# Autodesk Inventor assembly: Assembly6
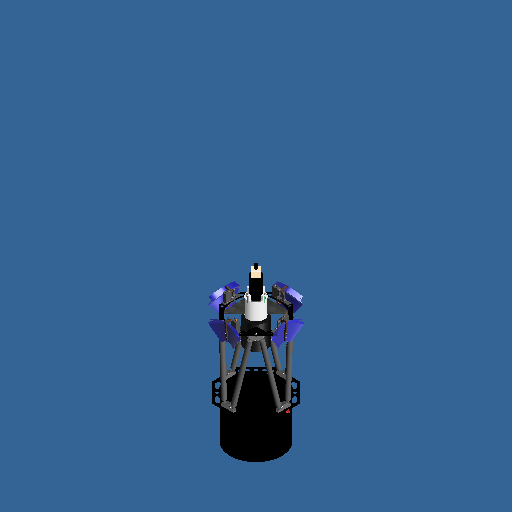
[picture p0: Inventor's stored thumbnail of the model, 512x512]
Saved by Autodesk Inventor 2026.2 (Build 302298000, 298)
## iProperties
Created: 2025-12-09
Part Number: Assembly6
Document SubType Name: Assembly
Designer: Thoma
Mass: 27295.5 g
Surface Area: 25498 cm^2
Volume: 10830.6 cm^3
Density: 2.52023 g/cm^3
Author: Thoma
## Documents named in this file (39)
- C:\Users\Thoma\OneDrive\Desktop\dir\telescope_cover\main\version_2\Main_v5.iam
- C:\Users\Thoma\OneDrive\Desktop\dir\telescope_cover\telescope\version_3\Telescope_End.ipt
- C:\Users\Thoma\OneDrive\Desktop\dir\telescope_cover\telescope\version_3\Triangle.ipt
- C:\Users\Thoma\OneDrive\Desktop\dir\telescope_cover\telescope\version_3\Triangle_Bracket_Top.ipt
- C:\Users\Thoma\OneDrive\Desktop\dir\telescope_cover\telescope\version_3\Carbon_Fibre.ipt
- C:\Users\Thoma\OneDrive\Desktop\dir\telescope_cover\telescope\version_3\5mm Screw.ipt
- C:\Users\Thoma\OneDrive\Desktop\dir\telescope_cover\telescope\version_3\35mm_bolt.ipt
- C:\Users\Thoma\OneDrive\Desktop\dir\telescope_cover\telescope\version_3\Triangle_Bracket_Bottom_MIR.ipt
- C:\Users\Thoma\OneDrive\Desktop\dir\telescope_cover\telescope\version_3\Telescope_Base.ipt
- C:\Users\Thoma\OneDrive\Desktop\dir\telescope_cover\telescope\version_3\Full_shaft_Simplify_3.ipt
- C:\Users\Thoma\OneDrive\Desktop\dir\telescope_cover\telescope\version_3\30mm_bolt.ipt
- C:\Users\Thoma\OneDrive\Desktop\dir\telescope_cover\telescope\version_3\Baffle.ipt
- C:\Users\Thoma\OneDrive\Desktop\dir\telescope_cover\telescope\version_3\Bottom_End_Top.ipt
- C:\Users\Thoma\OneDrive\Desktop\dir\telescope_cover\telescope\version_3\Laser.ipt
- C:\Users\Thoma\OneDrive\Desktop\dir\telescope_cover\cover\central_cover_v1.ipt
- C:\Users\Thoma\OneDrive\Desktop\dir\telescope_cover\cover\base_plate_v11.ipt
- C:\Users\Thoma\OneDrive\Desktop\dir\telescope_cover\cover\base_plate_bottom_v5.ipt
- C:\Users\Thoma\OneDrive\Documents\Inventor\Content Center Files\R2026\en-US\ISO 4035(2)\ISO 4035 - M4 - ISO.ipt
- C:\Users\Thoma\OneDrive\Desktop\dir\telescope_cover\servo\DSS-M15S Servo.ipt
- C:\Users\Thoma\OneDrive\Documents\Inventor\Content Center Files\R2026\en-US\ISO 4762(2)\ISO 4762 - M4 x 16ISO.ipt
- C:\Users\Thoma\OneDrive\Desktop\dir\telescope_cover\cover\pawn_v3.ipt
- C:\Users\Thoma\OneDrive\Documents\Inventor\Content Center Files\R2026\en-US\DIN 6796\DIN 6796 - 2.ipt
- C:\Users\Thoma\OneDrive\Documents\Inventor\Content Center Files\R2026\en-US\DIN 912\DIN 912 - M2 x 0.4 x 8 x 7.ipt
- C:\Users\Thoma\OneDrive\Documents\Inventor\Content Center Files\R2026\en-US\DIN 912\DIN 912 - M2 x 0.4 x 5 x 4.ipt
- C:\Users\Thoma\OneDrive\Desktop\dir\telescope_cover\cover\rod_v11.ipt
- C:\Users\Thoma\OneDrive\Documents\Inventor\Content Center Files\R2026\en-US\ISO 7092\ISO 7092 - ST 4 - 140 HV.ipt
- C:\Users\Thoma\OneDrive\Desktop\dir\telescope_cover\cover\Cover_Upper_v5.ipt
- C:\Users\Thoma\OneDrive\Desktop\dir\telescope_cover\cover\4mm_washer_1mm.ipt
- C:\Users\Thoma\OneDrive\Documents\Inventor\Content Center Files\R2026\en-US\ISO 4762(2)\ISO 4762 - M4 x 20ISO.ipt
- C:\Users\Thoma\OneDrive\Documents\Inventor\Content Center Files\R2026\en-US\ISO 4032(2)\ISO 4032 - M4 - ISO.ipt
- C:\Users\Thoma\OneDrive\Documents\Inventor\Content Center Files\R2026\en-US\ISO 7093 A\ISO 7093 A - ST 4 - 140 HV .ipt
- C:\Users\Thoma\OneDrive\Documents\Inventor\Content Center Files\R2026\en-US\ISO 4762(2)\ISO 4762 - M4 x 30ISO.ipt
- C:\Users\Thoma\OneDrive\Desktop\dir\telescope_cover\servo\limit_switch_v2.ipt
- C:\Users\Thoma\OneDrive\Documents\Inventor\Content Center Files\R2026\en-US\ISO 7089\ISO 7089 - 4 - 140 HV(1).ipt
- C:\Users\Thoma\OneDrive\Desktop\dir\telescope_cover\cover\base_plate_v12.ipt
- C:\Users\Thoma\OneDrive\Documents\Inventor\Content Center Files\R2026\en-US\ISO 7089\ISO 7089 - 2 - 140 HV(1).ipt
- C:\Users\Thoma\OneDrive\Documents\Inventor\Content Center Files\R2026\en-US\ISO 4762(2)\ISO 4762 - M2 x 8ISO.ipt
- C:\Users\Thoma\OneDrive\Desktop\dir\telescope_cover\cover\Cover_Lower_v5.ipt
- C:\Users\Thoma\OneDrive\Desktop\dir\telescope_cover\screws\M4 Washer - 9.0 x 0.9 - Black\M4 Washer - 9.0 x 0.9 - Black\M4 Washer - 9.0 x 0.9 - Black.ipt
## Components (238 placed, 38 different names)
1. Laser:2 — Mate:214, Flush:220, Flush:221
2. Laser:1 — Mate:215, Flush:218, Flush:219
3. Baffle:1 — Mate:83
4. Carbon_Fibre:1 — Mate:7, Mate:11, Flush:1, Mate:12, Mate:13, Mate:14, Mate:15, Mate:62, Mate:83, Mate:92, Mate:93, Mate:96, Mate:97, Mate:98, Mate:100, Mate:123, Mate:124, Mate:125, Mate:213, Mate:220, Angle:84, Flush:223, Flush:224, Flush:225, Flush:226
5. Telescope_Base:1 — Mate:62, Angle:31, Mate:89, Mate:90, Angle:40, Mate:108, Mate:109, Angle:48, Mate:110, Mate:111, Angle:49, Mate:112, Mate:113, Angle:50, Mate:214, Mate:215, Flush:218, Flush:221
6. Telescope_End:1 — Mate:1, Mate:2, Angle:2, Mate:7, Mate:54, Mate:55, Angle:26, Angle:31, Mate:86, Mate:88, Mate:91, Angle:41, Mate:101, Angle:45, Angle:46, Mate:114, Mate:115, Angle:51, Mate:116, Mate:117, Angle:52, Mate:118, Mate:119, Angle:53, Mate:229, Angle:85, Mate:230, Mate:231, Mate:332, Mate:333, Mate:334, Mate:335, Mate:336, Mate:337, Mate:341, Mate:342, Mate:344, Mate:345, Mate:346, Mate:347, Mate:362, Mate:378, Mate:421, Mate:422, Mate:423
7. 30mm_bolt:9 — Mate:217, Mate:218, Angle:83
8. 30mm_bolt:10 — Mate:216, Mate:219, Angle:82
9. Triangle_Bracket_Top:5 — Mate:116, Mate:117, Angle:52, Mate:129, Flush:110, Angle:60
10. Triangle_Bracket_Top:4 — Mate:101, Angle:45, Angle:46, Mate:104, Mate:105, Mate:106, Flush:103, Angle:47
11. Triangle_Bracket_Top:3 — Mate:86, Mate:88, Mate:94, Angle:54, Angle:55, Mate:122, Flush:106, Angle:56
12. Triangle_Bracket_Top:1 — Mate:1, Mate:2, Angle:2, Mate:8, Mate:9, Angle:4, Mate:47, Angle:22, Mate:58
13. 5mm Screw:14 — Mate:220, Flush:222, Angle:84
14. Triangle:1 — Mate:8, Mate:9, Angle:4, Mate:11, Flush:1, Angle:5, Angle:6, Mate:46, Mate:222, Mate:223
15. Triangle:5 — Mate:92, Mate:93, Mate:94, Mate:128, Flush:109, Angle:59, Flush:181, Angle:81, Mate:225, Mate:227
16. Triangle:6 — Mate:96, Mate:97, Mate:98, Flush:102, Angle:44, Mate:104, Mate:105, Flush:222, Mate:221, Mate:228
17. Triangle:7 — Mate:123, Mate:124, Mate:125, Mate:126, Flush:107, Angle:57, Mate:127, Flush:108, Angle:58, Mate:224, Mate:226
18. 35mm_bolt:6 — Mate:122, Flush:106, Angle:56
19. 35mm_bolt:7 — Mate:129, Flush:110, Angle:60
20. 35mm_bolt:4 — Mate:46, Mate:47, Angle:22
21. 35mm_bolt:5 — Mate:106, Flush:103, Angle:47
22. 5mm Screw:9 — Mate:100, Flush:102, Angle:44
23. 5mm Screw:13 — Mate:213, Flush:181, Angle:81
24. 5mm Screw:10 — Mate:126, Flush:107, Angle:57
25. 5mm Screw:2 — Mate:14, Mate:15, Angle:6
26. 5mm Screw:1 — Mate:12, Mate:13, Angle:5
27. 5mm Screw:11 — Mate:127, Flush:108, Angle:58
28. 5mm Screw:12 — Mate:128, Flush:109, Angle:59
29. Full_shaft_Simplify_3:1
30. Full_shaft_Simplify_3:2 — Tangent:26
31. Full_shaft_Simplify_3:3
32. Full_shaft_Simplify_3:4
33. Full_shaft_Simplify_3:5
34. Full_shaft_Simplify_3:6
35. Full_shaft_Simplify_3:7
36. Full_shaft_Simplify_3:8 — Tangent:31, Tangent:33
37. 30mm_bolt:7 — Mate:120, Flush:104, Angle:54
38. 30mm_bolt:1 — Mate:121, Flush:105, Angle:55
39. 30mm_bolt:8 — Mate:80, Flush:13, Angle:39
40. 30mm_bolt:6 — Mate:78, Flush:11, Angle:37
41. 30mm_bolt:3 — Mate:79, Flush:12, Angle:38
42. 30mm_bolt:2 — Mate:77, Flush:10, Angle:36
43. Triangle_Bracket_Bottom_MIR:4 — Mate:118, Mate:119, Angle:53, Mate:216, Mate:217, Mate:218, Mate:219, Angle:82, Angle:83
44. Triangle_Bracket_Bottom_MIR:3 — Mate:114, Mate:115, Angle:51, Mate:120, Flush:104, Mate:121, Flush:105
45. Triangle_Bracket_Bottom_MIR:2 — Mate:55, Mate:58, Angle:26, Mate:77, Flush:10, Angle:36, Mate:78, Flush:11, Angle:37, Tangent:31
46. Triangle_Bracket_Bottom_MIR:1 — Mate:54, Mate:79, Flush:12, Angle:38, Mate:80, Flush:13, Angle:39, Mate:91, Angle:41
47. Bottom_End_Top:4 — Mate:112, Mate:113, Angle:50, Tangent:26, Tangent:33
48. Bottom_End_Top:3 — Mate:110, Mate:111, Angle:49, Flush:219
49. Bottom_End_Top:2 — Mate:108, Mate:109, Angle:48
50. Bottom_End_Top:1 — Mate:89, Mate:90, Angle:40, Flush:220
51. central_cover_v1:1 — Mate:221, Mate:222, Flush:223, Mate:367, Mate:368, Mate:369
52. central_cover_v1:2 — Mate:223, Mate:224, Flush:224, Mate:375, Mate:376, Mate:381
53. central_cover_v1:3 — Mate:225, Mate:226, Flush:225, Mate:374, Mate:377, Mate:382
54. central_cover_v1:4 — Mate:227, Mate:228, Flush:226, Mate:372, Mate:373, Mate:383
55. limit_switch_v2:2 — Mate:370, Mate:371, Flush:227
56. limit_switch_v2:1 — Mate:367, Mate:368, Mate:369
57. base_plate_bottom_v5:5 — Mate:362, Mate:363, Mate:364, Mate:370, Mate:371, Flush:227
58. base_plate_v11:1 — Mate:229, Angle:85, Mate:230, Mate:231, Angle:92, Mate:262, Mate:263, Mate:264, Mate:271, Mate:272, Mate:273, Mate:274, Mate:275, Mate:276, Mate:277, Mate:278, Mate:282, Mate:307, Mate:308, Mate:309, Mate:310, Mate:312, Mate:314, Mate:320, Mate:321, Mate:322, Mate:324, Mate:325, Mate:326, Mate:328, Mate:329, Mate:330
59. pawn_v3:1 — Angle:92, Mate:281, Mate:282, Mate:311, Mate:313
60. DSS-M15S Servo:1 — Mate:262, Mate:263, Mate:264, Mate:279, Mate:280
61. DIN 6796 2:1 — Mate:271, Mate:272, Insert:6
62. DIN 912 - replaced by DIN EN ISO 4762 M2 x 8:1 — Insert:6
63. DIN 6796 2:2 — Mate:273, Mate:274, Insert:7
64. DIN 912 - replaced by DIN EN ISO 4762 M2 x 5:1 — Insert:7
65. DIN 6796 2:3 — Mate:275, Mate:276, Insert:8
66. DIN 912 - replaced by DIN EN ISO 4762 M2 x 8:2 — Insert:8
67. DIN 6796 2:4 — Mate:277, Mate:278, Insert:9
68. DIN 912 - replaced by DIN EN ISO 4762 M2 x 8:3 — Insert:9
69. rod_v11:1 — Mate:279, Mate:280, Mate:281, Mate:287, Mate:288, Tangent:34, Mate:289, Mate:290, Mate:291, Mate:292, Mate:293, Mate:294, Mate:295, Mate:297, Mate:298, Mate:299, Mate:301, Mate:302, Mate:303, Mate:305, Mate:306
70. Cover_Upper_v5:1 — Mate:287, Mate:288, Tangent:34, Mate:296, Mate:300, Mate:304
71. 4mm_washer_1mm:1 — Mate:289, Mate:294
72. 4mm_washer_1mm:2 — Mate:290, Mate:293
73. 4mm_washer_1mm:3 — Mate:291, Mate:292
74. ISO 7092 ST 4 - 140 HV:3 — Mate:295, Mate:296, Insert:12
75. ISO 4762 M4 x 16:3 — Insert:12
76. ISO 7092 ST 4 - 140 HV:4 — Mate:297, Mate:298, Insert:13
77. ISO 4035 M4:5 — Insert:13
78. ISO 7092 ST 4 - 140 HV:5 — Mate:299, Mate:300, Insert:14
79. ISO 4762 M4 x 16:4 — Insert:14
80. ISO 7092 ST 4 - 140 HV:6 — Mate:301, Mate:302, Insert:15
81. ISO 4035 M4:6 — Insert:15
82. ISO 7092 ST 4 - 140 HV:7 — Mate:303, Mate:304, Insert:16
83. ISO 4762 M4 x 16:5 — Insert:16
84. ISO 7092 ST 4 - 140 HV:8 — Mate:305, Mate:306, Insert:17
85. ISO 4035 M4:7 — Insert:17
86. ISO 4762 M4 x 20:1 — Mate:307, Mate:308
87. ISO 4035 M4:8 — Mate:309, Mate:310
88. ISO 4762 M4 x 20:2 — Mate:311, Mate:312
89. ISO 4035 M4:9 — Mate:313, Mate:314
90. ISO 7092 ST 4 - 140 HV:11 — Mate:320, Mate:321, Insert:20
91. ISO 4762 M4 x 20:4 — Insert:20
92. ISO 7093 A ST 4 - 140 HV - A:1 — Mate:322, Insert:21
93. ISO 4032 M4:2 — Insert:21
94. ISO 7092 ST 4 - 140 HV:12 — Mate:324, Mate:325, Insert:22
95. ISO 4762 M4 x 20:5 — Insert:22, Mate:363
96. ISO 7093 A ST 4 - 140 HV - A:2 — Mate:326, Insert:23
97. ISO 4032 M4:3 — Insert:23
98. ISO 7092 ST 4 - 140 HV:13 — Mate:328, Mate:329, Insert:24
99. ISO 4762 M4 x 30:1 — Insert:24, Mate:364
100. ISO 7093 A ST 4 - 140 HV - A:3 — Mate:330, Insert:25
101. ISO 4032 M4:4 — Insert:25
102. Cover_Lower_v5:1 — Mate:448, Mate:455, Tangent:35, Mate:456, Mate:457, Mate:458, Mate:461, Mate:465
103. M4 Washer - 9.0 x 0.9 - Black:1 — Mate:449, Mate:454, Tangent:35
104. M4 Washer - 9.0 x 0.9 - Black:2 — Mate:450, Mate:453
105. M4 Washer - 9.0 x 0.9 - Black:3 — Mate:451, Mate:452
106. ISO 7092 ST 4 - 140 HV:30 — Mate:456, Mate:457, Insert:50
107. ISO 4762 M4 x 20:15 — Insert:50
108. ISO 7089 4:2 — Mate:458, Mate:459, Insert:51
109. ISO 4032 M4:15 — Insert:51
110. ISO 7092 ST 4 - 140 HV:31 — Mate:460, Mate:461, Insert:52
111. ISO 4762 M4 x 20:16 — Insert:52
112. ISO 7089 4:3 — Mate:462, Mate:463, Insert:53
113. ISO 4032 M4:16 — Insert:53
114. ISO 7092 ST 4 - 140 HV:32 — Mate:464, Mate:465, Insert:54
115. ISO 4762 M4 x 20:17 — Insert:54
116. ISO 7089 4:4 — Mate:466, Mate:467, Insert:55
117. ISO 4032 M4:17 — Insert:55
118. DSS-M15S Servo:2 — Mate:435, Mate:436, Mate:437, Mate:446, Mate:447
119. ISO 7089 2:1 — Mate:438, Mate:439, Insert:46
120. ISO 4762 M2 x 8:1 — Insert:46
121. ISO 7089 2:2 — Mate:440, Mate:441, Insert:47
122. ISO 4762 M2 x 8:2 — Insert:47
123. ISO 7089 2:3 — Mate:442, Mate:443, Insert:48
124. ISO 4762 M2 x 8:3 — Insert:48
125. ISO 7089 2:4 — Mate:444, Mate:445, Insert:49
126. ISO 4762 M2 x 8:4 — Insert:49
127. rod_v11:2 — Mate:446, Mate:447, Mate:448, Mate:449, Mate:450, Mate:451, Mate:452, Mate:453, Mate:454, Mate:455, Mate:459, Mate:460, Mate:462, Mate:463, Mate:464, Mate:466, Mate:467
128. ISO 4762 M4 x 20:13 — Mate:427, Mate:428
129. ISO 4035 M4:10 — Mate:429, Mate:430
130. ISO 4762 M4 x 20:14 — Mate:431, Mate:432
131. ISO 4035 M4:11 — Mate:433, Mate:434
132. pawn_v3:2 — Mate:424, Mate:425, Mate:426, Mate:431, Mate:433
133. base_plate_v12:1 — Mate:421, Mate:422, Mate:423, Mate:424, Mate:425, Mate:426, Mate:427, Mate:428, Mate:429, Mate:430, Mate:432, Mate:434, Mate:435, Mate:436, Mate:437, Mate:438, Mate:439, Mate:440, Mate:441, Mate:442, Mate:443, Mate:444, Mate:445
134. limit_switch_v2:8 — Mate:388, Mate:389, Mate:390
135. limit_switch_v2:3 — Mate:372, Mate:373, Mate:383
136. ISO 7092 ST 4 - 140 HV:14 — Insert:26
137. ISO 4762 M4 x 30:2 — Insert:26
138. ISO 7093 A ST 4 - 140 HV - A:4 — Mate:353, Insert:27
139. ISO 4032 M4:5 — Insert:27
140. ISO 7092 ST 4 - 140 HV:15 — Insert:28
141. ISO 4762 M4 x 20:6 — Insert:28
142. ISO 7093 A ST 4 - 140 HV - A:5 — Mate:357, Insert:29
143. ISO 4032 M4:6 — Insert:29
144. base_plate_bottom_v5:2 — Mate:332, Mate:333, Mate:334, Mate:353, Mate:357, Mate:388, Mate:389, Mate:390
145. ISO 7092 ST 4 - 140 HV:36 — Mate:544, Mate:545, Insert:70
146. ISO 4762 M4 x 20:25 — Insert:70
147. ISO 7089 4:8 — Mate:546, Mate:547, Insert:71
148. ISO 4032 M4:21 — Insert:71
149. ISO 7092 ST 4 - 140 HV:37 — Mate:548, Mate:549, Insert:72
150. ISO 4762 M4 x 20:26 — Insert:72
151. ISO 7089 4:9 — Mate:550, Mate:551, Insert:73
152. ISO 4032 M4:22 — Insert:73
153. ISO 7092 ST 4 - 140 HV:38 — Mate:552, Mate:553, Insert:74
154. ISO 4762 M4 x 20:27 — Insert:74
155. ISO 7089 4:10 — Mate:554, Mate:555, Insert:75
156. ISO 4032 M4:23 — Insert:75
157. ISO 4762 M4 x 20:20 — Mate:488, Mate:489
158. ISO 4035 M4:14 — Mate:490, Mate:491
159. ISO 4762 M4 x 20:21 — Mate:492, Mate:493
160. ISO 4035 M4:15 — Mate:494, Mate:495
161. Cover_Upper_v5:2 — Mate:522, Mate:523, Tangent:36, Mate:545, Mate:549, Mate:552, Mate:553, Mate:554
162. rod_v11:4 — Mate:514, Mate:515, Mate:516, Mate:517, Mate:518, Mate:519, Mate:520, Mate:521, Mate:522, Mate:523, Mate:544, Mate:546, Mate:547, Mate:548, Mate:550, Mate:551, Mate:555
163. M4 Washer - 9.0 x 0.9 - Black:4 — Mate:518, Mate:519, Tangent:36
164. M4 Washer - 9.0 x 0.9 - Black:5 — Mate:517, Mate:520
165. M4 Washer - 9.0 x 0.9 - Black:6 — Mate:516, Mate:521
166. ISO 7089 2:5 — Mate:496, Mate:497, Insert:56
167. ISO 4762 M2 x 8:5 — Insert:56
168. ISO 7089 2:6 — Mate:498, Mate:499, Insert:57
169. ISO 4762 M2 x 8:6 — Insert:57
170. ISO 7089 2:7 — Mate:500, Mate:501, Insert:58
171. ISO 4762 M2 x 8:7 — Insert:58
172. ISO 7089 2:8 — Mate:502, Mate:503, Insert:59
173. ISO 4762 M2 x 8:8 — Insert:59
174. pawn_v3:3 — Mate:468, Mate:469, Mate:470
175. DSS-M15S Servo:3 — Mate:471, Mate:472, Mate:473, Mate:514, Mate:515
176. ISO 7092 ST 4 - 140 HV:23 — Mate:405, Mate:406, Insert:38
177. ISO 4762 M4 x 20:10 — Insert:38
178. ISO 7092 ST 4 - 140 HV:24 — Mate:407, Mate:408, Insert:39
179. ISO 4032 M4:11 — Insert:39
180. ISO 7092 ST 4 - 140 HV:25 — Mate:409, Mate:410, Insert:40
181. ISO 4762 M4 x 20:11 — Insert:40
182. ISO 7092 ST 4 - 140 HV:26 — Mate:411, Mate:412, Insert:41
183. ISO 4032 M4:12 — Insert:41
184. ISO 7092 ST 4 - 140 HV:27 — Mate:413, Mate:414, Insert:42
185. ISO 4762 M4 x 30:4 — Insert:42
186. ISO 7092 ST 4 - 140 HV:28 — Mate:415, Mate:416, Insert:43
187. ISO 4032 M4:13 — Insert:43
188. limit_switch_v2:7 — Mate:385, Mate:386, Mate:387
189. limit_switch_v2:5 — Mate:374, Mate:377, Mate:382
190. base_plate_v11:4 — Mate:342, Mate:346, Mate:347, Mate:405, Mate:406, Mate:407, Mate:409, Mate:410, Mate:411, Mate:413, Mate:414, Mate:415, Mate:468, Mate:469, Mate:470, Mate:471, Mate:472, Mate:473, Mate:488, Mate:489, Mate:490, Mate:491, Mate:492, Mate:493, Mate:494, Mate:495, Mate:496, Mate:497, Mate:498, Mate:499, Mate:500, Mate:501, Mate:502, Mate:503
191. base_plate_bottom_v5:4 — Mate:335, Mate:336, Mate:337, Mate:385, Mate:386, Mate:387, Mate:408, Mate:412, Mate:416
192. ISO 4762 M4 x 20:18 — Mate:480, Mate:481
193. ISO 4035 M4:12 — Mate:482, Mate:483
194. ISO 4762 M4 x 20:19 — Mate:484, Mate:485
195. ISO 4035 M4:13 — Mate:486, Mate:487
196. ISO 7092 ST 4 - 140 HV:33 — Mate:532, Mate:533, Insert:64
197. ISO 4762 M4 x 20:22 — Insert:64
198. ISO 7089 4:5 — Mate:534, Mate:535, Insert:65
199. ISO 4032 M4:18 — Insert:65
200. ISO 7092 ST 4 - 140 HV:34 — Mate:536, Mate:537, Insert:66
201. ISO 4762 M4 x 20:23 — Insert:66
202. ISO 7089 4:6 — Mate:538, Mate:539, Insert:67
203. ISO 4032 M4:19 — Insert:67
204. ISO 7092 ST 4 - 140 HV:35 — Mate:540, Mate:541, Insert:68
205. ISO 4762 M4 x 20:24 — Insert:68
206. ISO 7089 4:7 — Mate:542, Mate:543, Insert:69
207. ISO 4032 M4:20 — Insert:69
208. M4 Washer - 9.0 x 0.9 - Black:7 — Mate:526, Mate:527, Tangent:37
209. M4 Washer - 9.0 x 0.9 - Black:8 — Mate:525, Mate:528
210. M4 Washer - 9.0 x 0.9 - Black:9 — Mate:524, Mate:529
211. Cover_Lower_v5:2 — Mate:530, Mate:531, Tangent:37, Mate:532, Mate:533, Mate:534, Mate:537, Mate:541
212. rod_v11:3 — Mate:512, Mate:513, Mate:524, Mate:525, Mate:526, Mate:527, Mate:528, Mate:529, Mate:530, Mate:531, Mate:535, Mate:536, Mate:538, Mate:539, Mate:540, Mate:542, Mate:543
213. ISO 7089 2:9 — Mate:504, Mate:505, Insert:60
214. ISO 4762 M2 x 8:9 — Insert:60
215. ISO 7089 2:10 — Mate:506, Mate:507, Insert:61
216. ISO 4762 M2 x 8:10 — Insert:61
217. ISO 7089 2:11 — Mate:508, Mate:509, Insert:62
218. ISO 4762 M2 x 8:11 — Insert:62
219. ISO 7089 2:12 — Mate:510, Mate:511, Insert:63
220. ISO 4762 M2 x 8:12 — Insert:63
221. DSS-M15S Servo:4 — Mate:474, Mate:475, Mate:476, Mate:512, Mate:513
222. pawn_v3:4 — Mate:477, Mate:478, Mate:479
223. ISO 7092 ST 4 - 140 HV:29 — Mate:417, Mate:418, Insert:44
224. ISO 7089 4:1 — Mate:419, Mate:420, Insert:45
225. ISO 4762 M4 x 20:12 — Insert:44
226. ISO 4032 M4:14 — Insert:45
227. ISO 7092 ST 4 - 140 HV:19 — Mate:397, Mate:398, Insert:34
228. ISO 4762 M4 x 20:9 — Insert:34
229. ISO 7092 ST 4 - 140 HV:20 — Mate:399, Mate:400, Insert:35
230. ISO 4032 M4:9 — Insert:35
231. ISO 7092 ST 4 - 140 HV:21 — Mate:401, Mate:402, Insert:36
232. ISO 4762 M4 x 30:3 — Insert:36
233. ISO 7092 ST 4 - 140 HV:22 — Mate:403, Mate:404, Insert:37
234. ISO 4032 M4:10 — Insert:37
235. limit_switch_v2:6 — Mate:379, Mate:380, Mate:384
236. base_plate_bottom_v5:6 — Mate:378, Mate:379, Mate:380, Mate:384, Mate:391, Mate:392, Mate:400, Mate:404, Mate:420
237. limit_switch_v2:4 — Mate:375, Mate:376, Mate:381
238. base_plate_v11:2 — Mate:341, Mate:344, Mate:345, Mate:391, Mate:392, Mate:397, Mate:398, Mate:399, Mate:401, Mate:402, Mate:403, Mate:417, Mate:418, Mate:419, Mate:474, Mate:475, Mate:476, Mate:477, Mate:478, Mate:479, Mate:480, Mate:481, Mate:482, Mate:483, Mate:484, Mate:485, Mate:486, Mate:487, Mate:504, Mate:505, Mate:506, Mate:507, Mate:508, Mate:509, Mate:510, Mate:511
## Relationships (462: Mate 332, Insert 62, Angle 36, Flush 25, Tangent 7)
- Mate:1: Telescope_End:1 ↔ Triangle_Bracket_Top:1
- Mate:2: Telescope_End:1 ↔ Triangle_Bracket_Top:1
- Angle:2 (0 deg): Telescope_End:1 ↔ Triangle_Bracket_Top:1
- Mate:7: Carbon_Fibre:1 ↔ Telescope_End:1
- Mate:8: Triangle_Bracket_Top:1 ↔ Triangle:1
- Mate:9: Triangle_Bracket_Top:1 ↔ Triangle:1
- Angle:4 (0 deg): Triangle_Bracket_Top:1 ↔ Triangle:1
- Mate:11: Carbon_Fibre:1 ↔ Triangle:1
- Flush:1: Carbon_Fibre:1 ↔ Triangle:1
- Mate:12: Carbon_Fibre:1 ↔ 5mm Screw:1
- Mate:13: Carbon_Fibre:1 ↔ 5mm Screw:1
- Angle:5 (0 deg): Triangle:1 ↔ 5mm Screw:1
- Mate:14: Carbon_Fibre:1 ↔ 5mm Screw:2
- Mate:15: Carbon_Fibre:1 ↔ 5mm Screw:2
- Angle:6 (0 deg): Triangle:1 ↔ 5mm Screw:2
- Mate:46: Triangle:1 ↔ 35mm_bolt:4
- Mate:47: Triangle_Bracket_Top:1 ↔ 35mm_bolt:4
- Angle:22 (0 deg): Triangle_Bracket_Top:1 ↔ 35mm_bolt:4
- Mate:54: Telescope_End:1 ↔ Triangle_Bracket_Bottom_MIR:1
- Mate:55: Telescope_End:1 ↔ Triangle_Bracket_Bottom_MIR:2
- Mate:58: Triangle_Bracket_Top:1 ↔ Triangle_Bracket_Bottom_MIR:2
- Angle:26 (0 deg): Telescope_End:1 ↔ Triangle_Bracket_Bottom_MIR:2
- Mate:62: Carbon_Fibre:1 ↔ Telescope_Base:1
- Angle:31 (0 deg): Telescope_Base:1 ↔ Telescope_End:1
- Mate:77: 30mm_bolt:2 ↔ Triangle_Bracket_Bottom_MIR:2
- Flush:10: 30mm_bolt:2 ↔ Triangle_Bracket_Bottom_MIR:2
- Angle:36 (0 deg): 30mm_bolt:2 ↔ Triangle_Bracket_Bottom_MIR:2
- Mate:78: 30mm_bolt:6 ↔ Triangle_Bracket_Bottom_MIR:2
- Flush:11: 30mm_bolt:6 ↔ Triangle_Bracket_Bottom_MIR:2
- Angle:37 (0 deg): 30mm_bolt:6 ↔ Triangle_Bracket_Bottom_MIR:2
- Mate:79: 30mm_bolt:3 ↔ Triangle_Bracket_Bottom_MIR:1
- Flush:12: 30mm_bolt:3 ↔ Triangle_Bracket_Bottom_MIR:1
- Angle:38 (0 deg): 30mm_bolt:3 ↔ Triangle_Bracket_Bottom_MIR:1
- Mate:80: 30mm_bolt:8 ↔ Triangle_Bracket_Bottom_MIR:1
- Flush:13: 30mm_bolt:8 ↔ Triangle_Bracket_Bottom_MIR:1
- Angle:39 (0 deg): 30mm_bolt:8 ↔ Triangle_Bracket_Bottom_MIR:1
- Mate:83: Baffle:1 ↔ Carbon_Fibre:1
- Mate:86: Telescope_End:1 ↔ Triangle_Bracket_Top:3
- Mate:88: Telescope_End:1 ↔ Triangle_Bracket_Top:3
- Mate:89: Telescope_Base:1 ↔ Bottom_End_Top:1
- Mate:90: Telescope_Base:1 ↔ Bottom_End_Top:1
- Angle:40 (0 deg): Telescope_Base:1 ↔ Bottom_End_Top:1
- Mate:91: Telescope_End:1 ↔ Triangle_Bracket_Bottom_MIR:1
- Angle:41 (0 deg): Telescope_End:1 ↔ Triangle_Bracket_Bottom_MIR:1
- Mate:92: Carbon_Fibre:1 ↔ Triangle:5
- Mate:93: Carbon_Fibre:1 ↔ Triangle:5
- Mate:94: Triangle_Bracket_Top:3 ↔ Triangle:5
- Mate:96: Carbon_Fibre:1 ↔ Triangle:6
- Mate:97: Carbon_Fibre:1 ↔ Triangle:6
- Mate:98: Carbon_Fibre:1 ↔ Triangle:6
- Mate:100: Carbon_Fibre:1 ↔ 5mm Screw:9
- Flush:102: Triangle:6 ↔ 5mm Screw:9
- Angle:44 (0 deg): Triangle:6 ↔ 5mm Screw:9
- Mate:101: Telescope_End:1 ↔ Triangle_Bracket_Top:4
- Angle:45 (0 deg): Telescope_End:1 ↔ Triangle_Bracket_Top:4
- Angle:46 (0 deg): Telescope_End:1 ↔ Triangle_Bracket_Top:4
- Mate:104: Triangle_Bracket_Top:4 ↔ Triangle:6
- Mate:105: Triangle_Bracket_Top:4 ↔ Triangle:6
- Mate:106: Triangle_Bracket_Top:4 ↔ 35mm_bolt:5
- Flush:103: Triangle_Bracket_Top:4 ↔ 35mm_bolt:5
- Angle:47 (0 deg): Triangle_Bracket_Top:4 ↔ 35mm_bolt:5
- Mate:108: Telescope_Base:1 ↔ Bottom_End_Top:2
- Mate:109: Telescope_Base:1 ↔ Bottom_End_Top:2
- Angle:48 (0 deg): Telescope_Base:1 ↔ Bottom_End_Top:2
- Mate:110: Telescope_Base:1 ↔ Bottom_End_Top:3
- Mate:111: Telescope_Base:1 ↔ Bottom_End_Top:3
- Angle:49 (0 deg): Telescope_Base:1 ↔ Bottom_End_Top:3
- Mate:112: Telescope_Base:1 ↔ Bottom_End_Top:4
- Mate:113: Telescope_Base:1 ↔ Bottom_End_Top:4
- Angle:50 (0 deg): Telescope_Base:1 ↔ Bottom_End_Top:4
- Mate:114: Telescope_End:1 ↔ Triangle_Bracket_Bottom_MIR:3
- Mate:115: Telescope_End:1 ↔ Triangle_Bracket_Bottom_MIR:3
- Angle:51 (0 deg): Telescope_End:1 ↔ Triangle_Bracket_Bottom_MIR:3
- Mate:116: Telescope_End:1 ↔ Triangle_Bracket_Top:5
- Mate:117: Telescope_End:1 ↔ Triangle_Bracket_Top:5
- Angle:52 (0 deg): Telescope_End:1 ↔ Triangle_Bracket_Top:5
- Mate:118: Telescope_End:1 ↔ Triangle_Bracket_Bottom_MIR:4
- Mate:119: Telescope_End:1 ↔ Triangle_Bracket_Bottom_MIR:4
- Angle:53 (0 deg): Telescope_End:1 ↔ Triangle_Bracket_Bottom_MIR:4
- Mate:120: 30mm_bolt:7 ↔ Triangle_Bracket_Bottom_MIR:3
- Flush:104: 30mm_bolt:7 ↔ Triangle_Bracket_Bottom_MIR:3
- Angle:54 (0 deg): Triangle_Bracket_Top:3 ↔ 30mm_bolt:7
- Mate:121: 30mm_bolt:1 ↔ Triangle_Bracket_Bottom_MIR:3
- Flush:105: 30mm_bolt:1 ↔ Triangle_Bracket_Bottom_MIR:3
- Angle:55 (0 deg): Triangle_Bracket_Top:3 ↔ 30mm_bolt:1
- Mate:122: Triangle_Bracket_Top:3 ↔ 35mm_bolt:6
- Flush:106: Triangle_Bracket_Top:3 ↔ 35mm_bolt:6
- Angle:56 (0 deg): Triangle_Bracket_Top:3 ↔ 35mm_bolt:6
- Mate:123: Carbon_Fibre:1 ↔ Triangle:7
- Mate:124: Carbon_Fibre:1 ↔ Triangle:7
- Mate:125: Carbon_Fibre:1 ↔ Triangle:7
- Mate:126: Triangle:7 ↔ 5mm Screw:10
- Flush:107: Triangle:7 ↔ 5mm Screw:10
- Angle:57 (0 deg): Triangle:7 ↔ 5mm Screw:10
- Mate:127: Triangle:7 ↔ 5mm Screw:11
- Flush:108: Triangle:7 ↔ 5mm Screw:11
- Angle:58 (0 deg): Triangle:7 ↔ 5mm Screw:11
- Mate:128: Triangle:5 ↔ 5mm Screw:12
- Flush:109: Triangle:5 ↔ 5mm Screw:12
- Angle:59 (0 deg): Triangle:5 ↔ 5mm Screw:12
- Mate:129: Triangle_Bracket_Top:5 ↔ 35mm_bolt:7
- Flush:110: Triangle_Bracket_Top:5 ↔ 35mm_bolt:7
- Angle:60 (0 deg): Triangle_Bracket_Top:5 ↔ 35mm_bolt:7
- Mate:213: Carbon_Fibre:1 ↔ 5mm Screw:13
- Flush:181: Triangle:5 ↔ 5mm Screw:13
- Angle:81 (0 deg): Triangle:5 ↔ 5mm Screw:13
- Mate:214: Laser:2 ↔ Telescope_Base:1
- Mate:215: Laser:1 ↔ Telescope_Base:1
- Flush:218: Laser:1 ↔ Telescope_Base:1
- Flush:219 (39.316 mm): Laser:1 ↔ Bottom_End_Top:3
- Flush:220 (39.316 mm): Laser:2 ↔ Bottom_End_Top:1
- Flush:221: Laser:2 ↔ Telescope_Base:1
- Tangent:26: Full_shaft_Simplify_3:2 ↔ Bottom_End_Top:4
- Tangent:31: Full_shaft_Simplify_3:8 ↔ Triangle_Bracket_Bottom_MIR:2
- Tangent:33: Full_shaft_Simplify_3:8 ↔ Bottom_End_Top:4
- Mate:216: 30mm_bolt:10 ↔ Triangle_Bracket_Bottom_MIR:4
- Mate:217: 30mm_bolt:9 ↔ Triangle_Bracket_Bottom_MIR:4
- Mate:218: 30mm_bolt:9 ↔ Triangle_Bracket_Bottom_MIR:4
- Mate:219: 30mm_bolt:10 ↔ Triangle_Bracket_Bottom_MIR:4
- Angle:82 (0 deg): 30mm_bolt:10 ↔ Triangle_Bracket_Bottom_MIR:4
- Angle:83 (0 deg): 30mm_bolt:9 ↔ Triangle_Bracket_Bottom_MIR:4
- Mate:220: Carbon_Fibre:1 ↔ 5mm Screw:14
- Flush:222: 5mm Screw:14 ↔ Triangle:6
- Angle:84 (0 deg): Carbon_Fibre:1 ↔ 5mm Screw:14
- Mate:221: Triangle:6 ↔ central_cover_v1:1
- Mate:222: Triangle:1 ↔ central_cover_v1:1
- Flush:223: Carbon_Fibre:1 ↔ central_cover_v1:1
- Mate:223: Triangle:1 ↔ central_cover_v1:2
- Mate:224: Triangle:7 ↔ central_cover_v1:2
- Flush:224: Carbon_Fibre:1 ↔ central_cover_v1:2
- Mate:225: Triangle:5 ↔ central_cover_v1:3
- Mate:226: Triangle:7 ↔ central_cover_v1:3
- Flush:225: Carbon_Fibre:1 ↔ central_cover_v1:3
- Mate:227: Triangle:5 ↔ central_cover_v1:4
- Mate:228: Triangle:6 ↔ central_cover_v1:4
- Flush:226: Carbon_Fibre:1 ↔ central_cover_v1:4
- Mate:229: Telescope_End:1 ↔ base_plate_v11:1
- Angle:85 (0 deg): Telescope_End:1 ↔ base_plate_v11:1
- Mate:230: Telescope_End:1 ↔ base_plate_v11:1
- Mate:231: Telescope_End:1 ↔ base_plate_v11:1
- Angle:92 (0 deg): base_plate_v11:1 ↔ pawn_v3:1
- Mate:262: base_plate_v11:1 ↔ DSS-M15S Servo:1
- Mate:263 (1.1 mm): base_plate_v11:1 ↔ DSS-M15S Servo:1
- Mate:264: base_plate_v11:1 ↔ DSS-M15S Servo:1
- Mate:271: base_plate_v11:1 ↔ DIN 6796 2:1
- Mate:272: base_plate_v11:1 ↔ DIN 6796 2:1
- Insert:6: DIN 6796 2:1 ↔ DIN 912 - replaced by DIN EN ISO 4762 M2 x 8:1
- Mate:273: base_plate_v11:1 ↔ DIN 6796 2:2
- Mate:274: base_plate_v11:1 ↔ DIN 6796 2:2
- Insert:7: DIN 6796 2:2 ↔ DIN 912 - replaced by DIN EN ISO 4762 M2 x 5:1
- Mate:275: base_plate_v11:1 ↔ DIN 6796 2:3
- Mate:276: base_plate_v11:1 ↔ DIN 6796 2:3
- Insert:8: DIN 6796 2:3 ↔ DIN 912 - replaced by DIN EN ISO 4762 M2 x 8:2
- Mate:277: base_plate_v11:1 ↔ DIN 6796 2:4
- Mate:278: base_plate_v11:1 ↔ DIN 6796 2:4
- Insert:9: DIN 6796 2:4 ↔ DIN 912 - replaced by DIN EN ISO 4762 M2 x 8:3
- Mate:279: DSS-M15S Servo:1 ↔ rod_v11:1
- Mate:280: DSS-M15S Servo:1 ↔ rod_v11:1
- Mate:281: pawn_v3:1 ↔ rod_v11:1
- Mate:282 (0.4 mm): base_plate_v11:1 ↔ pawn_v3:1
- Mate:287: rod_v11:1 ↔ Cover_Upper_v5:1
- Mate:288: rod_v11:1 ↔ Cover_Upper_v5:1
- Tangent:34 (-1 mm): rod_v11:1 ↔ Cover_Upper_v5:1
- Mate:289: rod_v11:1 ↔ 4mm_washer_1mm:1
- Mate:290: rod_v11:1 ↔ 4mm_washer_1mm:2
- Mate:291: rod_v11:1 ↔ 4mm_washer_1mm:3
- Mate:292: rod_v11:1 ↔ 4mm_washer_1mm:3
- Mate:293: rod_v11:1 ↔ 4mm_washer_1mm:2
- Mate:294: rod_v11:1 ↔ 4mm_washer_1mm:1
- Mate:295: rod_v11:1 ↔ ISO 7092 ST 4 - 140 HV:3
- Mate:296: Cover_Upper_v5:1 ↔ ISO 7092 ST 4 - 140 HV:3
- Insert:12: ISO 7092 ST 4 - 140 HV:3 ↔ ISO 4762 M4 x 16:3
- Mate:297: rod_v11:1 ↔ ISO 7092 ST 4 - 140 HV:4
- Mate:298: rod_v11:1 ↔ ISO 7092 ST 4 - 140 HV:4
- Insert:13: ISO 7092 ST 4 - 140 HV:4 ↔ ISO 4035 M4:5
- Mate:299: rod_v11:1 ↔ ISO 7092 ST 4 - 140 HV:5
- Mate:300: Cover_Upper_v5:1 ↔ ISO 7092 ST 4 - 140 HV:5
- Insert:14: ISO 7092 ST 4 - 140 HV:5 ↔ ISO 4762 M4 x 16:4
- Mate:301: rod_v11:1 ↔ ISO 7092 ST 4 - 140 HV:6
- Mate:302: rod_v11:1 ↔ ISO 7092 ST 4 - 140 HV:6
- Insert:15: ISO 7092 ST 4 - 140 HV:6 ↔ ISO 4035 M4:6
- Mate:303: rod_v11:1 ↔ ISO 7092 ST 4 - 140 HV:7
- Mate:304: Cover_Upper_v5:1 ↔ ISO 7092 ST 4 - 140 HV:7
- Insert:16: ISO 7092 ST 4 - 140 HV:7 ↔ ISO 4762 M4 x 16:5
- Mate:305: rod_v11:1 ↔ ISO 7092 ST 4 - 140 HV:8
- Mate:306: rod_v11:1 ↔ ISO 7092 ST 4 - 140 HV:8
- Insert:17: ISO 7092 ST 4 - 140 HV:8 ↔ ISO 4035 M4:7
- Mate:307: base_plate_v11:1 ↔ ISO 4762 M4 x 20:1
- Mate:308: base_plate_v11:1 ↔ ISO 4762 M4 x 20:1
- Mate:309: base_plate_v11:1 ↔ ISO 4035 M4:8
- Mate:310: base_plate_v11:1 ↔ ISO 4035 M4:8
- Mate:311: pawn_v3:1 ↔ ISO 4762 M4 x 20:2
- Mate:312: base_plate_v11:1 ↔ ISO 4762 M4 x 20:2
- Mate:313: pawn_v3:1 ↔ ISO 4035 M4:9
- Mate:314: base_plate_v11:1 ↔ ISO 4035 M4:9
- Mate:320: base_plate_v11:1 ↔ ISO 7092 ST 4 - 140 HV:11
- Mate:321: base_plate_v11:1 ↔ ISO 7092 ST 4 - 140 HV:11
- Insert:20: ISO 7092 ST 4 - 140 HV:11 ↔ ISO 4762 M4 x 20:4
- Mate:322: base_plate_v11:1 ↔ ISO 7093 A ST 4 - 140 HV - A:1
- Insert:21: ISO 7093 A ST 4 - 140 HV - A:1 ↔ ISO 4032 M4:2
- Mate:324: base_plate_v11:1 ↔ ISO 7092 ST 4 - 140 HV:12
- Mate:325: base_plate_v11:1 ↔ ISO 7092 ST 4 - 140 HV:12
- Insert:22: ISO 7092 ST 4 - 140 HV:12 ↔ ISO 4762 M4 x 20:5
- Mate:326: base_plate_v11:1 ↔ ISO 7093 A ST 4 - 140 HV - A:2
- Insert:23: ISO 7093 A ST 4 - 140 HV - A:2 ↔ ISO 4032 M4:3
- Mate:328: base_plate_v11:1 ↔ ISO 7092 ST 4 - 140 HV:13
- Mate:329: base_plate_v11:1 ↔ ISO 7092 ST 4 - 140 HV:13
- Insert:24: ISO 7092 ST 4 - 140 HV:13 ↔ ISO 4762 M4 x 30:1
- Mate:330: base_plate_v11:1 ↔ ISO 7093 A ST 4 - 140 HV - A:3
- Insert:25: ISO 7093 A ST 4 - 140 HV - A:3 ↔ ISO 4032 M4:4
- Mate:332: Telescope_End:1 ↔ base_plate_bottom_v5:2
- Mate:333: Telescope_End:1 ↔ base_plate_bottom_v5:2
- Mate:334: Telescope_End:1 ↔ base_plate_bottom_v5:2
- Mate:335: Telescope_End:1 ↔ base_plate_bottom_v5:4
- Mate:336: Telescope_End:1 ↔ base_plate_bottom_v5:4
- Mate:337: Telescope_End:1 ↔ base_plate_bottom_v5:4
- Mate:341: Telescope_End:1 ↔ base_plate_v11:2
- Mate:342: Telescope_End:1 ↔ base_plate_v11:4
- Mate:344: Telescope_End:1 ↔ base_plate_v11:2
- Mate:345: Telescope_End:1 ↔ base_plate_v11:2
- Mate:346: Telescope_End:1 ↔ base_plate_v11:4
- Mate:347: Telescope_End:1 ↔ base_plate_v11:4
- Insert:26: ISO 7092 ST 4 - 140 HV:14 ↔ ISO 4762 M4 x 30:2
- Mate:353: ISO 7093 A ST 4 - 140 HV - A:4 ↔ base_plate_bottom_v5:2
- Insert:27: ISO 7093 A ST 4 - 140 HV - A:4 ↔ ISO 4032 M4:5
- Insert:28: ISO 7092 ST 4 - 140 HV:15 ↔ ISO 4762 M4 x 20:6
- Mate:357: ISO 7093 A ST 4 - 140 HV - A:5 ↔ base_plate_bottom_v5:2
- Insert:29: ISO 7093 A ST 4 - 140 HV - A:5 ↔ ISO 4032 M4:6
- Mate:362: Telescope_End:1 ↔ base_plate_bottom_v5:5
- Mate:363: base_plate_bottom_v5:5 ↔ ISO 4762 M4 x 20:5
- Mate:364: base_plate_bottom_v5:5 ↔ ISO 4762 M4 x 30:1
- Mate:367 (0.4 mm): central_cover_v1:1 ↔ limit_switch_v2:1
- Mate:368 (0.4 mm): central_cover_v1:1 ↔ limit_switch_v2:1
- Mate:369 (-17.1 mm): central_cover_v1:1 ↔ limit_switch_v2:1
- Mate:370 (0.4 mm): limit_switch_v2:2 ↔ base_plate_bottom_v5:5
- Mate:371 (0.4 mm): limit_switch_v2:2 ↔ base_plate_bottom_v5:5
- Flush:227: limit_switch_v2:2 ↔ base_plate_bottom_v5:5
- Mate:372 (0.4 mm): central_cover_v1:4 ↔ limit_switch_v2:3
- Mate:373 (0.4 mm): central_cover_v1:4 ↔ limit_switch_v2:3
- Mate:374: central_cover_v1:3 ↔ limit_switch_v2:5
- Mate:375 (0.4 mm): central_cover_v1:2 ↔ limit_switch_v2:4
- Mate:376 (0.4 mm): central_cover_v1:2 ↔ limit_switch_v2:4
- Mate:377: central_cover_v1:3 ↔ limit_switch_v2:5
- Mate:378: Telescope_End:1 ↔ base_plate_bottom_v5:6
- Mate:379 (0.4 mm): limit_switch_v2:6 ↔ base_plate_bottom_v5:6
- Mate:380 (0.4 mm): limit_switch_v2:6 ↔ base_plate_bottom_v5:6
- Mate:381 (-17.1 mm): central_cover_v1:2 ↔ limit_switch_v2:4
- Mate:382 (-17.1 mm): central_cover_v1:3 ↔ limit_switch_v2:5
- Mate:383 (-17.1 mm): central_cover_v1:4 ↔ limit_switch_v2:3
- Mate:384 (-15.1 mm): limit_switch_v2:6 ↔ base_plate_bottom_v5:6
- Mate:385 (0.4 mm): limit_switch_v2:7 ↔ base_plate_bottom_v5:4
- Mate:386 (0.4 mm): limit_switch_v2:7 ↔ base_plate_bottom_v5:4
- Mate:387 (-15.1 mm): limit_switch_v2:7 ↔ base_plate_bottom_v5:4
- Mate:388 (0.4 mm): limit_switch_v2:8 ↔ base_plate_bottom_v5:2
- Mate:389 (0.4 mm): limit_switch_v2:8 ↔ base_plate_bottom_v5:2
- Mate:390 (-15.1 mm): limit_switch_v2:8 ↔ base_plate_bottom_v5:2
- Mate:391: base_plate_bottom_v5:6 ↔ base_plate_v11:2
- Mate:392: base_plate_bottom_v5:6 ↔ base_plate_v11:2
- Mate:397: ISO 7092 ST 4 - 140 HV:19 ↔ base_plate_v11:2
- Mate:398: ISO 7092 ST 4 - 140 HV:19 ↔ base_plate_v11:2
- Insert:34: ISO 7092 ST 4 - 140 HV:19 ↔ ISO 4762 M4 x 20:9
- Mate:399: ISO 7092 ST 4 - 140 HV:20 ↔ base_plate_v11:2
- Mate:400: ISO 7092 ST 4 - 140 HV:20 ↔ base_plate_bottom_v5:6
- Insert:35: ISO 7092 ST 4 - 140 HV:20 ↔ ISO 4032 M4:9
- Mate:401: ISO 7092 ST 4 - 140 HV:21 ↔ base_plate_v11:2
- Mate:402: ISO 7092 ST 4 - 140 HV:21 ↔ base_plate_v11:2
- Insert:36: ISO 7092 ST 4 - 140 HV:21 ↔ ISO 4762 M4 x 30:3
- Mate:403: ISO 7092 ST 4 - 140 HV:22 ↔ base_plate_v11:2
- Mate:404: ISO 7092 ST 4 - 140 HV:22 ↔ base_plate_bottom_v5:6
- Insert:37: ISO 7092 ST 4 - 140 HV:22 ↔ ISO 4032 M4:10
- Mate:405: ISO 7092 ST 4 - 140 HV:23 ↔ base_plate_v11:4
- Mate:406: ISO 7092 ST 4 - 140 HV:23 ↔ base_plate_v11:4
- Insert:38: ISO 7092 ST 4 - 140 HV:23 ↔ ISO 4762 M4 x 20:10
- Mate:407: ISO 7092 ST 4 - 140 HV:24 ↔ base_plate_v11:4
- Mate:408: ISO 7092 ST 4 - 140 HV:24 ↔ base_plate_bottom_v5:4
- Insert:39: ISO 7092 ST 4 - 140 HV:24 ↔ ISO 4032 M4:11
- Mate:409: ISO 7092 ST 4 - 140 HV:25 ↔ base_plate_v11:4
- Mate:410: ISO 7092 ST 4 - 140 HV:25 ↔ base_plate_v11:4
- Insert:40: ISO 7092 ST 4 - 140 HV:25 ↔ ISO 4762 M4 x 20:11
- Mate:411: ISO 7092 ST 4 - 140 HV:26 ↔ base_plate_v11:4
- Mate:412: ISO 7092 ST 4 - 140 HV:26 ↔ base_plate_bottom_v5:4
- Insert:41: ISO 7092 ST 4 - 140 HV:26 ↔ ISO 4032 M4:12
- Mate:413: ISO 7092 ST 4 - 140 HV:27 ↔ base_plate_v11:4
- Mate:414: ISO 7092 ST 4 - 140 HV:27 ↔ base_plate_v11:4
- Insert:42: ISO 7092 ST 4 - 140 HV:27 ↔ ISO 4762 M4 x 30:4
- Mate:415: ISO 7092 ST 4 - 140 HV:28 ↔ base_plate_v11:4
- Mate:416: ISO 7092 ST 4 - 140 HV:28 ↔ base_plate_bottom_v5:4
- Insert:43: ISO 7092 ST 4 - 140 HV:28 ↔ ISO 4032 M4:13
- Mate:417: ISO 7092 ST 4 - 140 HV:29 ↔ base_plate_v11:2
- Mate:418: ISO 7092 ST 4 - 140 HV:29 ↔ base_plate_v11:2
- Insert:44: ISO 7092 ST 4 - 140 HV:29 ↔ ISO 4762 M4 x 20:12
- Mate:419: ISO 7089 4:1 ↔ base_plate_v11:2
- Mate:420: ISO 7089 4:1 ↔ base_plate_bottom_v5:6
- Insert:45: ISO 7089 4:1 ↔ ISO 4032 M4:14
- Mate:421: Telescope_End:1 ↔ base_plate_v12:1
- Mate:422: Telescope_End:1 ↔ base_plate_v12:1
- Mate:423: Telescope_End:1 ↔ base_plate_v12:1
- Mate:424: pawn_v3:2 ↔ base_plate_v12:1
- Mate:425: pawn_v3:2 ↔ base_plate_v12:1
- Mate:426 (0.4 mm): pawn_v3:2 ↔ base_plate_v12:1
- Mate:427: ISO 4762 M4 x 20:13 ↔ base_plate_v12:1
- Mate:428: ISO 4762 M4 x 20:13 ↔ base_plate_v12:1
- Mate:429: ISO 4035 M4:10 ↔ base_plate_v12:1
- Mate:430: ISO 4035 M4:10 ↔ base_plate_v12:1
- Mate:431: ISO 4762 M4 x 20:14 ↔ pawn_v3:2
- Mate:432: ISO 4762 M4 x 20:14 ↔ base_plate_v12:1
- Mate:433: ISO 4035 M4:11 ↔ pawn_v3:2
- Mate:434: ISO 4035 M4:11 ↔ base_plate_v12:1
- Mate:435: DSS-M15S Servo:2 ↔ base_plate_v12:1
- Mate:436 (1.1 mm): DSS-M15S Servo:2 ↔ base_plate_v12:1
- Mate:437: DSS-M15S Servo:2 ↔ base_plate_v12:1
- Mate:438: ISO 7089 2:1 ↔ base_plate_v12:1
- Mate:439: ISO 7089 2:1 ↔ base_plate_v12:1
- Insert:46: ISO 7089 2:1 ↔ ISO 4762 M2 x 8:1
- Mate:440: ISO 7089 2:2 ↔ base_plate_v12:1
- Mate:441: ISO 7089 2:2 ↔ base_plate_v12:1
- Insert:47: ISO 7089 2:2 ↔ ISO 4762 M2 x 8:2
- Mate:442: ISO 7089 2:3 ↔ base_plate_v12:1
- Mate:443: ISO 7089 2:3 ↔ base_plate_v12:1
- Insert:48: ISO 7089 2:3 ↔ ISO 4762 M2 x 8:3
- Mate:444: ISO 7089 2:4 ↔ base_plate_v12:1
- Mate:445: ISO 7089 2:4 ↔ base_plate_v12:1
- Insert:49: ISO 7089 2:4 ↔ ISO 4762 M2 x 8:4
- Mate:446: DSS-M15S Servo:2 ↔ rod_v11:2
- Mate:447: DSS-M15S Servo:2 ↔ rod_v11:2
- Mate:448: Cover_Lower_v5:1 ↔ rod_v11:2
- Mate:449: M4 Washer - 9.0 x 0.9 - Black:1 ↔ rod_v11:2
- Mate:450: M4 Washer - 9.0 x 0.9 - Black:2 ↔ rod_v11:2
- Mate:451: M4 Washer - 9.0 x 0.9 - Black:3 ↔ rod_v11:2
- Mate:452: M4 Washer - 9.0 x 0.9 - Black:3 ↔ rod_v11:2
- Mate:453: M4 Washer - 9.0 x 0.9 - Black:2 ↔ rod_v11:2
- Mate:454: M4 Washer - 9.0 x 0.9 - Black:1 ↔ rod_v11:2
- Mate:455: Cover_Lower_v5:1 ↔ rod_v11:2
- Tangent:35: Cover_Lower_v5:1 ↔ M4 Washer - 9.0 x 0.9 - Black:1
- Mate:456: Cover_Lower_v5:1 ↔ ISO 7092 ST 4 - 140 HV:30
- Mate:457: Cover_Lower_v5:1 ↔ ISO 7092 ST 4 - 140 HV:30
- Insert:50: ISO 7092 ST 4 - 140 HV:30 ↔ ISO 4762 M4 x 20:15
- Mate:458: Cover_Lower_v5:1 ↔ ISO 7089 4:2
- Mate:459: ISO 7089 4:2 ↔ rod_v11:2
- Insert:51: ISO 7089 4:2 ↔ ISO 4032 M4:15
- Mate:460: ISO 7092 ST 4 - 140 HV:31 ↔ rod_v11:2
- Mate:461: Cover_Lower_v5:1 ↔ ISO 7092 ST 4 - 140 HV:31
- Insert:52: ISO 7092 ST 4 - 140 HV:31 ↔ ISO 4762 M4 x 20:16
- Mate:462: ISO 7089 4:3 ↔ rod_v11:2
- Mate:463: ISO 7089 4:3 ↔ rod_v11:2
- Insert:53: ISO 7089 4:3 ↔ ISO 4032 M4:16
- Mate:464: ISO 7092 ST 4 - 140 HV:32 ↔ rod_v11:2
- Mate:465: Cover_Lower_v5:1 ↔ ISO 7092 ST 4 - 140 HV:32
- Insert:54: ISO 7092 ST 4 - 140 HV:32 ↔ ISO 4762 M4 x 20:17
- Mate:466: ISO 7089 4:4 ↔ rod_v11:2
- Mate:467: ISO 7089 4:4 ↔ rod_v11:2
- Insert:55: ISO 7089 4:4 ↔ ISO 4032 M4:17
- Mate:468: pawn_v3:3 ↔ base_plate_v11:4
- Mate:469: pawn_v3:3 ↔ base_plate_v11:4
- Mate:470 (0.4 mm): pawn_v3:3 ↔ base_plate_v11:4
- Mate:471: DSS-M15S Servo:3 ↔ base_plate_v11:4
- Mate:472 (1.1 mm): DSS-M15S Servo:3 ↔ base_plate_v11:4
- Mate:473: DSS-M15S Servo:3 ↔ base_plate_v11:4
- Mate:474: DSS-M15S Servo:4 ↔ base_plate_v11:2
- Mate:475 (1.1 mm): DSS-M15S Servo:4 ↔ base_plate_v11:2
- Mate:476: DSS-M15S Servo:4 ↔ base_plate_v11:2
- Mate:477: pawn_v3:4 ↔ base_plate_v11:2
- Mate:478: pawn_v3:4 ↔ base_plate_v11:2
- Mate:479 (0.4 mm): pawn_v3:4 ↔ base_plate_v11:2
- Mate:480: ISO 4762 M4 x 20:18 ↔ base_plate_v11:2
- Mate:481: ISO 4762 M4 x 20:18 ↔ base_plate_v11:2
- Mate:482: ISO 4035 M4:12 ↔ base_plate_v11:2
- Mate:483: ISO 4035 M4:12 ↔ base_plate_v11:2
- Mate:484: ISO 4762 M4 x 20:19 ↔ base_plate_v11:2
- Mate:485: ISO 4762 M4 x 20:19 ↔ base_plate_v11:2
- Mate:486: ISO 4035 M4:13 ↔ base_plate_v11:2
- Mate:487: ISO 4035 M4:13 ↔ base_plate_v11:2
- Mate:488: ISO 4762 M4 x 20:20 ↔ base_plate_v11:4
- Mate:489: ISO 4762 M4 x 20:20 ↔ base_plate_v11:4
- Mate:490: ISO 4035 M4:14 ↔ base_plate_v11:4
- Mate:491: ISO 4035 M4:14 ↔ base_plate_v11:4
- Mate:492: ISO 4762 M4 x 20:21 ↔ base_plate_v11:4
- Mate:493: ISO 4762 M4 x 20:21 ↔ base_plate_v11:4
- Mate:494: ISO 4035 M4:15 ↔ base_plate_v11:4
- Mate:495: ISO 4035 M4:15 ↔ base_plate_v11:4
- Mate:496: ISO 7089 2:5 ↔ base_plate_v11:4
- Mate:497: ISO 7089 2:5 ↔ base_plate_v11:4
- Insert:56: ISO 7089 2:5 ↔ ISO 4762 M2 x 8:5
- Mate:498: ISO 7089 2:6 ↔ base_plate_v11:4
- Mate:499: ISO 7089 2:6 ↔ base_plate_v11:4
- Insert:57: ISO 7089 2:6 ↔ ISO 4762 M2 x 8:6
- Mate:500: ISO 7089 2:7 ↔ base_plate_v11:4
- Mate:501: ISO 7089 2:7 ↔ base_plate_v11:4
- Insert:58: ISO 7089 2:7 ↔ ISO 4762 M2 x 8:7
- Mate:502: ISO 7089 2:8 ↔ base_plate_v11:4
- Mate:503: ISO 7089 2:8 ↔ base_plate_v11:4
- Insert:59: ISO 7089 2:8 ↔ ISO 4762 M2 x 8:8
- Mate:504: ISO 7089 2:9 ↔ base_plate_v11:2
- Mate:505: ISO 7089 2:9 ↔ base_plate_v11:2
- Insert:60: ISO 7089 2:9 ↔ ISO 4762 M2 x 8:9
- Mate:506: ISO 7089 2:10 ↔ base_plate_v11:2
- Mate:507: ISO 7089 2:10 ↔ base_plate_v11:2
- Insert:61: ISO 7089 2:10 ↔ ISO 4762 M2 x 8:10
- Mate:508: ISO 7089 2:11 ↔ base_plate_v11:2
- Mate:509: ISO 7089 2:11 ↔ base_plate_v11:2
- Insert:62: ISO 7089 2:11 ↔ ISO 4762 M2 x 8:11
- Mate:510: ISO 7089 2:12 ↔ base_plate_v11:2
- Mate:511: ISO 7089 2:12 ↔ base_plate_v11:2
- Insert:63: ISO 7089 2:12 ↔ ISO 4762 M2 x 8:12
- Mate:512: rod_v11:3 ↔ DSS-M15S Servo:4
- Mate:513: rod_v11:3 ↔ DSS-M15S Servo:4
- Mate:514: rod_v11:4 ↔ DSS-M15S Servo:3
- Mate:515: rod_v11:4 ↔ DSS-M15S Servo:3
- Mate:516: rod_v11:4 ↔ M4 Washer - 9.0 x 0.9 - Black:6
- Mate:517: rod_v11:4 ↔ M4 Washer - 9.0 x 0.9 - Black:5
- Mate:518: rod_v11:4 ↔ M4 Washer - 9.0 x 0.9 - Black:4
- Mate:519: rod_v11:4 ↔ M4 Washer - 9.0 x 0.9 - Black:4
- Mate:520: rod_v11:4 ↔ M4 Washer - 9.0 x 0.9 - Black:5
- Mate:521: rod_v11:4 ↔ M4 Washer - 9.0 x 0.9 - Black:6
- Mate:522: Cover_Upper_v5:2 ↔ rod_v11:4
- Mate:523: Cover_Upper_v5:2 ↔ rod_v11:4
- Tangent:36: Cover_Upper_v5:2 ↔ M4 Washer - 9.0 x 0.9 - Black:4
- Mate:524: M4 Washer - 9.0 x 0.9 - Black:9 ↔ rod_v11:3
- Mate:525: M4 Washer - 9.0 x 0.9 - Black:8 ↔ rod_v11:3
- Mate:526: M4 Washer - 9.0 x 0.9 - Black:7 ↔ rod_v11:3
- Mate:527: M4 Washer - 9.0 x 0.9 - Black:7 ↔ rod_v11:3
- Mate:528: M4 Washer - 9.0 x 0.9 - Black:8 ↔ rod_v11:3
- Mate:529: M4 Washer - 9.0 x 0.9 - Black:9 ↔ rod_v11:3
- Mate:530: Cover_Lower_v5:2 ↔ rod_v11:3
- Mate:531: Cover_Lower_v5:2 ↔ rod_v11:3
- Tangent:37: M4 Washer - 9.0 x 0.9 - Black:7 ↔ Cover_Lower_v5:2
- Mate:532: ISO 7092 ST 4 - 140 HV:33 ↔ Cover_Lower_v5:2
- Mate:533: ISO 7092 ST 4 - 140 HV:33 ↔ Cover_Lower_v5:2
- Insert:64: ISO 7092 ST 4 - 140 HV:33 ↔ ISO 4762 M4 x 20:22
- Mate:534: ISO 7089 4:5 ↔ Cover_Lower_v5:2
- Mate:535: ISO 7089 4:5 ↔ rod_v11:3
- Insert:65: ISO 7089 4:5 ↔ ISO 4032 M4:18
- Mate:536: ISO 7092 ST 4 - 140 HV:34 ↔ rod_v11:3
- Mate:537: ISO 7092 ST 4 - 140 HV:34 ↔ Cover_Lower_v5:2
- Insert:66: ISO 7092 ST 4 - 140 HV:34 ↔ ISO 4762 M4 x 20:23
- Mate:538: ISO 7089 4:6 ↔ rod_v11:3
- Mate:539: ISO 7089 4:6 ↔ rod_v11:3
- Insert:67: ISO 7089 4:6 ↔ ISO 4032 M4:19
- Mate:540: ISO 7092 ST 4 - 140 HV:35 ↔ rod_v11:3
- Mate:541: ISO 7092 ST 4 - 140 HV:35 ↔ Cover_Lower_v5:2
- Insert:68: ISO 7092 ST 4 - 140 HV:35 ↔ ISO 4762 M4 x 20:24
- Mate:542: ISO 7089 4:7 ↔ rod_v11:3
- Mate:543: ISO 7089 4:7 ↔ rod_v11:3
- Insert:69: ISO 7089 4:7 ↔ ISO 4032 M4:20
- Mate:544: ISO 7092 ST 4 - 140 HV:36 ↔ rod_v11:4
- Mate:545: ISO 7092 ST 4 - 140 HV:36 ↔ Cover_Upper_v5:2
- Insert:70: ISO 7092 ST 4 - 140 HV:36 ↔ ISO 4762 M4 x 20:25
- Mate:546: ISO 7089 4:8 ↔ rod_v11:4
- Mate:547: ISO 7089 4:8 ↔ rod_v11:4
- Insert:71: ISO 7089 4:8 ↔ ISO 4032 M4:21
- Mate:548: ISO 7092 ST 4 - 140 HV:37 ↔ rod_v11:4
- Mate:549: ISO 7092 ST 4 - 140 HV:37 ↔ Cover_Upper_v5:2
- Insert:72: ISO 7092 ST 4 - 140 HV:37 ↔ ISO 4762 M4 x 20:26
- Mate:550: ISO 7089 4:9 ↔ rod_v11:4
- Mate:551: ISO 7089 4:9 ↔ rod_v11:4
- Insert:73: ISO 7089 4:9 ↔ ISO 4032 M4:22
- Mate:552: ISO 7092 ST 4 - 140 HV:38 ↔ Cover_Upper_v5:2
- Mate:553: ISO 7092 ST 4 - 140 HV:38 ↔ Cover_Upper_v5:2
- Insert:74: ISO 7092 ST 4 - 140 HV:38 ↔ ISO 4762 M4 x 20:27
- Mate:554: ISO 7089 4:10 ↔ Cover_Upper_v5:2
- Mate:555: ISO 7089 4:10 ↔ rod_v11:4
- Insert:75: ISO 7089 4:10 ↔ ISO 4032 M4:23
